# Autodesk Inventor assembly: robot
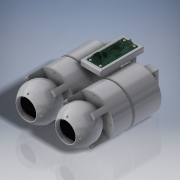
[picture p0: Inventor's stored thumbnail of the model, 180x180]
Saved by Autodesk Inventor 2016 (Build 200138000, 138)
## iProperties
Created: 2017-09-19
Part Number: robot
Document SubType Name: Assembly
Designer: Hamid
Author: Hamid
## Documents named in this file (10)
- C:\Users\Hamid Osooli\Desktop\BSc Project\3D Plans\robot.iam
- C:\Users\Hamid Osooli\Desktop\BSc Project\3D Plans\camera.ipt
- C:\Users\Hamid Osooli\Desktop\BSc Project\3D Plans\eye ball cap.ipt
- C:\Users\Hamid Osooli\Desktop\BSc Project\3D Plans\eye ball.ipt
- C:\Users\Hamid Osooli\Desktop\BSc Project\3D Plans\left_orbit.ipt
- C:\Users\Hamid Osooli\Desktop\BSc Project\3D Plans\servo.ipt
- C:\Users\Hamid Osooli\Desktop\BSc Project\3D Plans\back orbit.ipt
- C:\Users\Hamid Osooli\Desktop\BSc Project\3D Plans\right_rorbit.ipt
- C:\Users\Hamid Osooli\Desktop\BSc Project\3D Plans\handle2.ipt
- C:\Users\Hamid Osooli\Desktop\BSc Project\3D Plans\opencm.ipt
## Components (16 placed, 9 different names)
1. camera:1 — Insert:1, Insert:6
2. eye ball cap:1 — Insert:2
3. eye ball:1 — Insert:1, Insert:2
4. left_orbit:1 — Insert:3, Insert:5, Insert:6
5. servo:1 — Insert:3
6. back orbit:1 — Insert:4, Insert:5, Insert:14
7. servo:3 — Insert:4
8. camera:2 — Insert:13
9. eye ball cap:2
10. eye ball:2
11. servo:4 — Insert:11
12. back orbit:2 — Insert:12, Insert:15
13. servo:5
14. right_rorbit:1 — Insert:11, Insert:12, Insert:13
15. handle2:2 — Insert:14, Insert:15
16. opencm:1
## Relationships (14: Insert 14)
- Insert:1 (-27.432 mm): camera:1 ↔ eye ball:1
- Insert:2 (-5.08 mm): eye ball cap:1 ↔ eye ball:1
- Insert:3 (-24.13 mm): left_orbit:1 ↔ servo:1
- Insert:4 (-24.13 mm): back orbit:1 ↔ servo:3
- Insert:5 (-7.62 mm): left_orbit:1 ↔ back orbit:1
- Insert:6 (17.018 mm): camera:1 ↔ left_orbit:1
- [Insert] (-27.432 mm): camera:2 ↔ eye ball:2
- [Insert] (-5.08 mm): eye ball cap:2 ↔ eye ball:2
- [Insert] (-24.13 mm): back orbit:2 ↔ servo:5
- Insert:11 (-24.13 mm): servo:4 ↔ right_rorbit:1
- Insert:12 (-7.62 mm): back orbit:2 ↔ right_rorbit:1
- Insert:13 (17.018 mm): camera:2 ↔ right_rorbit:1
- Insert:14: back orbit:1 ↔ handle2:2
- Insert:15: back orbit:2 ↔ handle2:2
## Named parameters: d8_d4 = -24.13 mm, d11_d1 = -5.08 mm, d12_d0 = -27.432 mm
